# Autodesk Inventor assembly: 8233K16_Aluminum Round Turntable
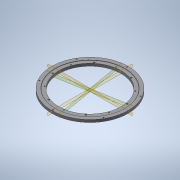
[picture p0: Inventor's stored thumbnail of the model, 180x180]
Saved by Autodesk Inventor 2020 (Build 240168000, 168)
## iProperties
Created: 2022-02-23
Part Number: 8233K16_Aluminum Round Turntable
Document SubType Name: Assembly
Designer: mavericks
Author: mavericks
## Documents named in this file (3)
- T:\EIT\2022 Rapid React\COMMON PARTS\MCMASTER\8233K16_Aluminum Round Turntable.iam
- T:\EIT\2022 Rapid React\COMMON PARTS\MCMASTER\Solid1_1.ipt
- T:\EIT\2022 Rapid React\COMMON PARTS\MCMASTER\Solid14.ipt
## Components (2 placed, 2 different names)
1. Solid1_1:1 — Mate:1, Flush:1
2. Solid14:1 — Mate:1, Flush:1
## Relationships (2: Mate 1, Flush 1)
- Mate:1: Solid1_1:1 ↔ Solid14:1
- Flush:1 (-0.9906 mm): Solid1_1:1 ↔ Solid14:1
